# Autodesk Inventor assembly: Gestikulaser
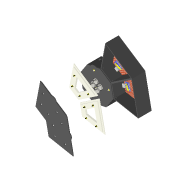
[picture p0: Inventor's stored thumbnail of the model, 180x180]
Saved by Autodesk Inventor 2018.2 (Build 222227000, 227)
## iProperties
Created: 2018-11-01
Part Number: Gestikulaser
Material: Generisch
Document SubType Name: Assembly
Designer: M.Knabel
Author: M.Knabel
## Documents named in this file (3)
- V:\A340\2018\DOKUMENTATION\COSIMA\COSIMA-Laserstar\CAD\Gestikulaser.iam
- V:\A340\2018\DOKUMENTATION\COSIMA\COSIMA-Laserstar\CAD\Oktokommander\Oktokommander.iam
- V:\A340\2018\DOKUMENTATION\COSIMA\COSIMA-Laserstar\CAD\Detektormodul\Detektormodul.iam
## Components (7 placed, 2 different names)
1. Detektormodul:2 [sub-assembly] — Passend:1, Fluchtend:2, Passend:4
2. Detektormodul:3 [sub-assembly] — Fluchtend:2, Fluchtend:3, Passend:3, Passend:5
3. Detektormodul:5 [sub-assembly]
4. Detektormodul:6 [sub-assembly]
5. Detektormodul:7 [sub-assembly]
6. Detektormodul:8 [sub-assembly] — Fluchtend:1, Passend:2
7. Oktokommander:1 [sub-assembly] — Fluchtend:1, Passend:1, Passend:2, Fluchtend:3, Passend:3, Passend:4, Passend:5, Passend:6, Passend:7, Passend:8
## Relationships (11: Mate 8, Flush 3)
- Fluchtend:1 [Flush]: Detektormodul:8 ↔ Oktokommander:1
- Passend:1 [Mate]: Detektormodul:2 ↔ Oktokommander:1
- Passend:2 [Mate]: Detektormodul:8 ↔ Oktokommander:1
- Fluchtend:2 [Flush]: Detektormodul:2 ↔ Detektormodul:3
- Fluchtend:3 [Flush]: Detektormodul:3 ↔ Oktokommander:1
- Passend:3 [Mate]: Detektormodul:3 ↔ Oktokommander:1
- Passend:4 [Mate]: Detektormodul:2 ↔ Oktokommander:1
- Passend:5 [Mate]: Detektormodul:3 ↔ Oktokommander:1
- Passend:6 [Mate]: Oktokommander:1
- Passend:7 [Mate]: Oktokommander:1
- Passend:8 [Mate]: Oktokommander:1
